# Autodesk Inventor assembly: inner_assy
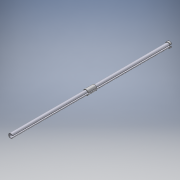
[picture p0: Inventor's stored thumbnail of the model, 180x180]
Saved by Autodesk Inventor 2017 (Build 210142000, 142)
## iProperties
Created: 2018-11-30
Part Number: inner_assy
Document SubType Name: Assembly
Designer: ddeboer
Author: ddeboer
## Documents named in this file (5)
- C:\Users\ddeboer\Desktop\sch40_conduit\inner_assy.iam
- C:\Users\ddeboer\Desktop\sch40_conduit\inner_sheath.ipt
- C:\Users\ddeboer\Desktop\sch40_conduit\coupler.ipt
- C:\Users\ddeboer\Desktop\sch40_conduit\ring.ipt
- C:\Users\ddeboer\Desktop\sch40_conduit\inner_extender.ipt
## Components (4 placed, 4 different names)
1. inner_sheath:1 — Insert:1, Insert:2, Insert:3
2. coupler:1 — Insert:1
3. ring:1 — Insert:2
4. inner_extender:1 — Insert:3
## Relationships (3: Insert 3)
- Insert:1 (26 mm): inner_sheath:1 ↔ coupler:1
- Insert:2: inner_sheath:1 ↔ ring:1
- Insert:3: inner_sheath:1 ↔ inner_extender:1
